# Autodesk Inventor assembly: CNC-A-ASSEMBLY
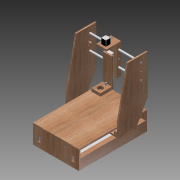
[picture p0: Inventor's stored thumbnail of the model, 180x180]
Saved by Autodesk Inventor 2015 (Build 190159000, 159)
## iProperties
Created: 2015-03-25
Part Number: CNC-A-ASSEMBLY
Document SubType Name: Assembly
Designer: Bangladesh
Author: Bangladesh
## Documents named in this file (5)
- C:\Users\Alvi\Documents\CNC design files\Assemblies\CNC-A-ASSEMBLY.iam
- C:\Users\Alvi\Documents\CNC design files\Assemblies\CNC-X-axis- ASSEMBLY.iam
- C:\Users\Alvi\Documents\CNC design files\Assemblies\CNC-Y-axis- ASSEMBLY.iam
- C:\Users\Alvi\Documents\CNC design files\CNC-A- Y-axis support on X-axis.ipt
- C:\Users\Alvi\Documents\CNC design files\Assemblies\CNC-Z-axis- ASSEMBLY.iam
## Components (5 placed, 4 different names)
1. CNC-X-axis- ASSEMBLY:1 [sub-assembly] — Mate:4, Mate:5, Mate:6, Mate:8, Mate:10
2. CNC-Y-axis- ASSEMBLY:1 [sub-assembly] — Mate:4, Mate:5, Mate:6, Mate:7, Mate:9, Rotational:1
3. CNC-A- Y-axis support on X-axis:1 — Mate:9, Mate:10
4. CNC-A- Y-axis support on X-axis:2 — Mate:7, Mate:8
5. CNC-Z-axis- ASSEMBLY:1 [sub-assembly] — Rotational:1
## Relationships (8: Mate 7, RevoluteJoint 1)
- Mate:4: CNC-X-axis- ASSEMBLY:1 ↔ CNC-Y-axis- ASSEMBLY:1
- Mate:5: CNC-X-axis- ASSEMBLY:1 ↔ CNC-Y-axis- ASSEMBLY:1
- Mate:6: CNC-X-axis- ASSEMBLY:1 ↔ CNC-Y-axis- ASSEMBLY:1
- Mate:7: CNC-Y-axis- ASSEMBLY:1 ↔ CNC-A- Y-axis support on X-axis:2
- Mate:8: CNC-X-axis- ASSEMBLY:1 ↔ CNC-A- Y-axis support on X-axis:2
- Mate:9: CNC-Y-axis- ASSEMBLY:1 ↔ CNC-A- Y-axis support on X-axis:1
- Mate:10: CNC-X-axis- ASSEMBLY:1 ↔ CNC-A- Y-axis support on X-axis:1
- Rotational:1 [RevoluteJoint] (9.525 mm): CNC-Y-axis- ASSEMBLY:1 ↔ CNC-Z-axis- ASSEMBLY:1
